# Autodesk Inventor assembly: gear
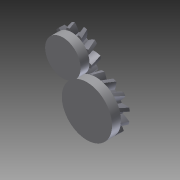
[picture p0: Inventor's stored thumbnail of the model, 180x180]
Saved by Autodesk Inventor 2012 (Build 160160000, 160)
## iProperties
Created: 2011-10-26
Part Number: gear
Document SubType Name: Assembly
Designer: akutta
Author: akutta
## Documents named in this file (4)
- C:\Users\akutta\Documents\gear.iam
- C:\Users\akutta\Documents\gear1.ipt
- C:\Users\akutta\Documents\gear2.ipt
- C:\Users\akutta\Documents\gear\Design Accelerator\Spur Gears1.iam
## Components (3 placed, 3 different names)
1. gear1:1 — Flush:1, Mate:1, Mate:4, Mate:5
2. gear2:1 — Flush:1, Mate:1, Mate:2, Mate:3
3. Spur Gears:1 [sub-assembly] — Mate:2, Mate:3, Mate:4, Mate:5
## Relationships (6: Mate 5, Flush 1)
- Flush:1: gear1:1 ↔ gear2:1
- Mate:1 (18.72 mm): gear1:1 ↔ gear2:1
- Mate:2: gear2:1 ↔ Spur Gears:1
- Mate:3: gear2:1 ↔ Spur Gears:1
- Mate:4: gear1:1 ↔ Spur Gears:1
- Mate:5: gear1:1 ↔ Spur Gears:1
